# Autodesk Inventor assembly: Assembly3
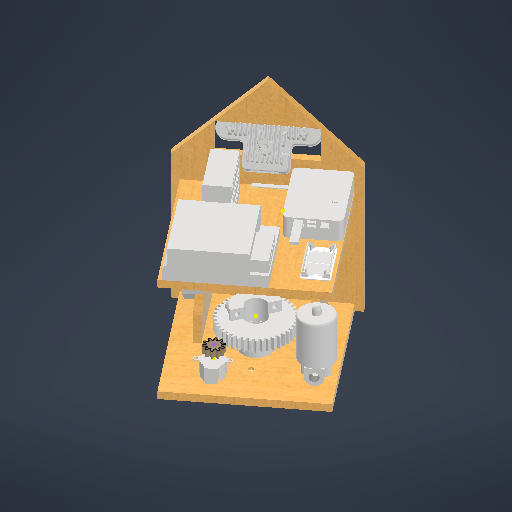
[picture p0: Inventor's stored thumbnail of the model, 512x512]
Saved by Autodesk Inventor 2026.2 (Build 302298000, 298)
## iProperties
Created: 2026-01-14
Part Number: Assembly3
Document SubType Name: Assembly
Designer: User
Author: User
## Documents named in this file (23)
- C:\Users\User\Classes\Capstone\3d\redesign but smaller\Assembly3.iam
- C:\Users\User\Classes\Capstone\3d\redesign but smaller\pole_v2.ipt
- C:\Users\User\Classes\Capstone\3d\redesign but smaller\birdhouse_holder_v1.ipt
- C:\Users\User\Classes\Capstone\3d\redesign but smaller\605_2rs_bearing.ipt
- C:\Users\User\Classes\Capstone\3d\redesign but smaller\pole_ring_v1_with_clamp.ipt
- C:\Users\User\Classes\Capstone\3d\redesign but smaller\base_plate.ipt
- C:\Users\User\Classes\Capstone\3d\redesign but smaller\drive_gear_v1.ipt
- C:\Users\User\Classes\Capstone\3d\redesign but smaller\stepper_motor.ipt
- C:\Users\User\Classes\Capstone\3d\redesign but smaller\side wall.ipt
- C:\Users\User\Classes\Capstone\3d\redesign but smaller\front wall.ipt
- C:\Users\User\Classes\Capstone\3d\redesign but smaller\turret_lift.ipt
- C:\Users\User\Classes\Capstone\3d\redesign but smaller\bearing_holder_v2_left.ipt
- C:\Users\User\Classes\Capstone\3d\redesign but smaller\bearing_holder_v2_right.ipt
- C:\Users\User\Classes\Capstone\3d\redesign but smaller\pitch_motor_standoff_v1.ipt
- C:\Users\User\Classes\Capstone\3d\redesign but smaller\pitch gear v3.ipt
- C:\Users\User\Classes\Capstone\3d\redesign but smaller\temp_nozzle_v2.ipt
- C:\Users\User\Classes\Capstone\3d\redesign but smaller\pole_gear_v3_with_clamp.ipt
- C:\Users\User\Classes\Capstone\3d\redesign but smaller\ElectronicValve.ipt
- C:\Users\User\Classes\Capstone\3d\redesign but smaller\RaspberryPi.ipt
- C:\Users\User\Classes\Capstone\3d\redesign but smaller\PowerSupply.ipt
- C:\Users\User\Classes\Capstone\3d\redesign but smaller\Relay.ipt
- C:\Users\User\Classes\Capstone\3d\redesign but smaller\Camera_v2.ipt
- C:\Users\User\Classes\Capstone\3d\redesign but smaller\relay board holder.ipt
## Components (29 placed, 22 different names)
1. pole_v2:1 — Mate:2, Mate:8, Mate:52, Flush:25, Flush:26
2. birdhouse_holder_v1:1 — Mate:2, Mate:4, Mate:5, Mate:6, Mate:7, Mate:11, Mate:12, Mate:13
3. 605_2rs_bearing:1 — Mate:6, Mate:7
4. 605_2rs_bearing:2 — Mate:4, Mate:5, Tangent:1
5. pole_ring_v1_with_clamp:3 — Mate:8, Tangent:1, Angle:3
6. base_plate:1 — Mate:11, Mate:12, Mate:13, Flush:4, Flush:5, Mate:16, Flush:6, Flush:7, Mate:17, Flush:9, Mate:21, Flush:26, Mate:53, Mate:55, Flush:27, Flush:28, Mate:56, Flush:29, Flush:30
7. drive_gear_v1:1 — Mate:14, Mate:15
8. stepper_motor:1 — Mate:14, Mate:15, Flush:4, Flush:5, Mate:53
9. side wall:1 — Mate:16, Flush:6, Flush:7, Flush:8, Mate:18
10. front wall:1 — Mate:17, Flush:8, Flush:9, Mate:20, Angle:7, Mate:63, Flush:41, Mate:68
11. turret_lift:1 — Mate:18, Mate:19, Flush:10, Flush:11, Mate:20, Mate:22, Flush:12, Mate:23, Mate:26, Mate:28, Angle:2
12. turret_lift:2 — Mate:19, Flush:10, Flush:11, Mate:21, Mate:24, Flush:13, Mate:25, Mate:27
13. bearing_holder_v2_left:1 — Mate:22, Flush:12, Mate:23, Mate:34, Mate:35
14. bearing_holder_v2_right:1 — Mate:24, Flush:13, Mate:25
15. pitch_motor_standoff_v1:1 — Mate:26, Mate:27, Mate:28, Mate:29, Mate:30, Angle:1
16. stepper_motor:2 — Mate:29, Mate:30, Angle:1, Mate:31, Mate:54
17. drive_gear_v1:2 — Mate:31, Mate:54
18. pitch gear v3:1 — Mate:34, Mate:35, Angle:2, Mate:36, Flush:14, Mate:37
19. temp_nozzle_v2:1 — Mate:36, Flush:14, Mate:37
20. pole_gear_v3_with_clamp:1 — Mate:52, Angle:3, Flush:25
21. ElectronicValve:1 — Mate:55, Flush:27, Flush:28
22. base_plate:2 — Mate:56, Flush:29, Flush:30, Mate:59, Angle:6, Angle:8, Mate:67, Flush:46, Mate:69, Flush:47, Flush:48, Flush:49, Mate:71, Flush:50, Flush:51
23. PowerSupply:1 — Mate:69, Flush:47, Flush:48, Mate:70
24. Relay:1 — Mate:59, Mate:60, Flush:33, Angle:6, Flush:45, Mate:70, Flush:49
25. Relay:2 — Mate:60, Mate:61, Flush:32, Flush:33, Flush:34, Flush:45
26. Relay:3 — Mate:61, Flush:32, Flush:34
27. Camera_v2:1 — Angle:7, Angle:8, Mate:63, Flush:41
28. RaspberryPi:1 — Mate:67, Flush:46, Mate:68
29. relay board holder:1 — Mate:71, Flush:50, Flush:51
## Relationships (80: Mate 45, Flush 28, Angle 6, Tangent 1)
- Mate:2: pole_v2:1 ↔ birdhouse_holder_v1:1
- Mate:4: birdhouse_holder_v1:1 ↔ 605_2rs_bearing:2
- Mate:5: birdhouse_holder_v1:1 ↔ 605_2rs_bearing:2
- Mate:6: birdhouse_holder_v1:1 ↔ 605_2rs_bearing:1
- Mate:7: birdhouse_holder_v1:1 ↔ 605_2rs_bearing:1
- Mate:8: pole_v2:1 ↔ pole_ring_v1_with_clamp:3
- Tangent:1: 605_2rs_bearing:2 ↔ pole_ring_v1_with_clamp:3
- Mate:11: birdhouse_holder_v1:1 ↔ base_plate:1
- Mate:12: birdhouse_holder_v1:1 ↔ base_plate:1
- Mate:13: birdhouse_holder_v1:1 ↔ base_plate:1
- Mate:14: drive_gear_v1:1 ↔ stepper_motor:1
- Mate:15: drive_gear_v1:1 ↔ stepper_motor:1
- Flush:4 (20 mm): base_plate:1 ↔ stepper_motor:1
- Flush:5 (120 mm): base_plate:1 ↔ stepper_motor:1
- Mate:16: base_plate:1 ↔ side wall:1
- Flush:6: base_plate:1 ↔ side wall:1
- Flush:7: base_plate:1 ↔ side wall:1
- Mate:17: base_plate:1 ↔ front wall:1
- Flush:8: side wall:1 ↔ front wall:1
- Flush:9: base_plate:1 ↔ front wall:1
- Mate:18 (25 mm): side wall:1 ↔ turret_lift:1
- Mate:19 (110 mm): turret_lift:1 ↔ turret_lift:2
- Flush:10: turret_lift:1 ↔ turret_lift:2
- Flush:11: turret_lift:1 ↔ turret_lift:2
- Mate:20: front wall:1 ↔ turret_lift:1
- Mate:21: base_plate:1 ↔ turret_lift:2
- Mate:22: turret_lift:1 ↔ bearing_holder_v2_left:1
- Flush:12: turret_lift:1 ↔ bearing_holder_v2_left:1
- Mate:23: turret_lift:1 ↔ bearing_holder_v2_left:1
- Mate:24: turret_lift:2 ↔ bearing_holder_v2_right:1
- Flush:13: turret_lift:2 ↔ bearing_holder_v2_right:1
- Mate:25: turret_lift:2 ↔ bearing_holder_v2_right:1
- Mate:26: turret_lift:1 ↔ pitch_motor_standoff_v1:1
- Mate:27: turret_lift:2 ↔ pitch_motor_standoff_v1:1
- Mate:28 (50 mm): turret_lift:1 ↔ pitch_motor_standoff_v1:1
- Mate:29: pitch_motor_standoff_v1:1 ↔ stepper_motor:2
- Mate:30: pitch_motor_standoff_v1:1 ↔ stepper_motor:2
- Angle:1 (180 deg): pitch_motor_standoff_v1:1 ↔ stepper_motor:2
- Mate:31: stepper_motor:2 ↔ drive_gear_v1:2
- Mate:34: bearing_holder_v2_left:1 ↔ pitch gear v3:1
- Mate:35: bearing_holder_v2_left:1 ↔ pitch gear v3:1
- Angle:2 (90 deg): turret_lift:1 ↔ pitch gear v3:1
- Mate:36: pitch gear v3:1 ↔ temp_nozzle_v2:1
- Flush:14: pitch gear v3:1 ↔ temp_nozzle_v2:1
- Mate:37 (-5 mm): pitch gear v3:1 ↔ temp_nozzle_v2:1
- Mate:52: pole_v2:1 ↔ pole_gear_v3_with_clamp:1
- Angle:3 (0 deg): pole_ring_v1_with_clamp:3 ↔ pole_gear_v3_with_clamp:1
- Flush:25: pole_v2:1 ↔ pole_gear_v3_with_clamp:1
- Flush:26 (53 mm): pole_v2:1 ↔ base_plate:1
- Mate:53: base_plate:1 ↔ stepper_motor:1
- Mate:54: stepper_motor:2 ↔ drive_gear_v1:2
- Mate:55: base_plate:1 ↔ ElectronicValve:1
- Flush:27 (30 mm): base_plate:1 ↔ ElectronicValve:1
- Flush:28 (12 mm): base_plate:1 ↔ ElectronicValve:1
- Mate:56 (130 mm): base_plate:1 ↔ base_plate:2
- Flush:29: base_plate:1 ↔ base_plate:2
- Flush:30: base_plate:1 ↔ base_plate:2
- Mate:59: base_plate:2 ↔ Relay:1
- Mate:60: Relay:1 ↔ Relay:2
- Mate:61: Relay:2 ↔ Relay:3
- Flush:32: Relay:2 ↔ Relay:3
- Flush:33: Relay:1 ↔ Relay:2
- Flush:34: Relay:2 ↔ Relay:3
- Angle:6 (90 deg): base_plate:2 ↔ Relay:1
- Angle:7 (-40 deg): front wall:1 ↔ Camera_v2:1
- Angle:8 (0 deg): base_plate:2 ↔ Camera_v2:1
- Mate:63: front wall:1 ↔ Camera_v2:1
- Flush:41 (100 mm): front wall:1 ↔ Camera_v2:1
- Flush:45: Relay:1 ↔ Relay:2
- Mate:67: base_plate:2 ↔ RaspberryPi:1
- Flush:46: base_plate:2 ↔ RaspberryPi:1
- Mate:68: front wall:1 ↔ RaspberryPi:1
- Mate:69: base_plate:2 ↔ PowerSupply:1
- Flush:47: base_plate:2 ↔ PowerSupply:1
- Flush:48 (5 mm): base_plate:2 ↔ PowerSupply:1
- Mate:70: PowerSupply:1 ↔ Relay:1
- Flush:49 (-35 mm): base_plate:2 ↔ Relay:1
- Mate:71: base_plate:2 ↔ relay board holder:1
- Flush:50 (5 mm): base_plate:2 ↔ relay board holder:1
- Flush:51 (20 mm): base_plate:2 ↔ relay board holder:1
